# Autodesk Inventor assembly: ideal_diode_ideal-diode
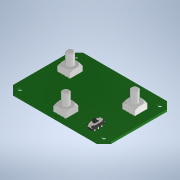
[picture p0: Inventor's stored thumbnail of the model, 180x180]
Saved by Autodesk Inventor 2021 (Build 250183000, 183)
## iProperties
Company: A Company
Created: 2021-01-31
Part Number: ideal_diode_ideal-diode
Description: KiCad electronic assembly
Document SubType Name: Assembly
Designer: oskar
Authority: Unknown
Sending System: KiCad to STEP converter
Preprocessor: Open CASCADE STEP processor 6.9
Title: ideal-diode.step
Author: An Author
## Documents named in this file (9)
- C:\Users\oskar\Dropbox\Dokument\Projekt\Elita\Electrical system\Highside-Powerdistribution\hardware\ideal-diode\cad\ideal_diode_ideal-diode.iam
- C:\Users\oskar\Dropbox\Dokument\Projekt\Elita\Electrical system\Highside-Powerdistribution\hardware\ideal-diode\cad\ideal_diode_D_SMB.iam
- C:\Users\oskar\Dropbox\Dokument\Projekt\Elita\Electrical system\Highside-Powerdistribution\hardware\ideal-diode\cad\ideal_diode_SW_CuK_JS202011CQN_DPDT_Straight.iam
- C:\Users\oskar\Dropbox\Dokument\Projekt\Elita\Electrical system\Highside-Powerdistribution\hardware\ideal-diode\cad\ideal_diode_M5_7461383_rev1.iam
- C:\Users\oskar\Dropbox\Dokument\Projekt\Elita\Electrical system\Highside-Powerdistribution\hardware\ideal-diode\cad\ideal_diode_SOT-23-6.iam
- C:\Users\oskar\Dropbox\Dokument\Projekt\Elita\Electrical system\Highside-Powerdistribution\hardware\ideal-diode\cad\ideal_diode_C_0603_1608Metric.iam
- C:\Users\oskar\Dropbox\Dokument\Projekt\Elita\Electrical system\Highside-Powerdistribution\hardware\ideal-diode\cad\ideal_diode_PowerPAK_SO-8L_SINGLE.iam
- C:\Users\oskar\Dropbox\Dokument\Projekt\Elita\Electrical system\Highside-Powerdistribution\hardware\ideal-diode\cad\ideal_diode_R_0603_1608Metric.iam
- C:\Users\oskar\Dropbox\Dokument\Projekt\Elita\Electrical system\Highside-Powerdistribution\hardware\ideal-diode\cad\ideal_diode_COMPOUND_1.ipt
## Components (14 placed, 14 different names)
1. 2 [sub-assembly]
2. 3 [sub-assembly]
3. 5 [sub-assembly] — Mate:1
4. 7 [sub-assembly]
5. 9 [sub-assembly]
6. 11 [sub-assembly]
7. 12 [sub-assembly]
8. 13 [sub-assembly]
9. 15 [sub-assembly]
10. 16 [sub-assembly]
11. 18 [sub-assembly]
12. 19 [sub-assembly]
13. 20 [sub-assembly]
14. 21 — Mate:1
## Relationships (1: Mate 1)
- Mate:1: 5 ↔ 21
